# Autodesk Inventor assembly: parts assembly
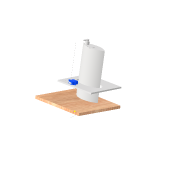
[picture p0: Inventor's stored thumbnail of the model, 180x180]
Saved by Autodesk Inventor 2021 (Build 250183000, 183)
## iProperties
Created: 2021-03-10
Part Number: parts assembly
Document SubType Name: Assembly
Designer: Dell
Author: Dell
## Documents named in this file (8)
- D:\project\parts assembly.iam
- D:\project\base.ipt
- D:\project\ir.ipt
- D:\project\Servo Motor SG90.ipt
- D:\project\arm.ipt
- D:\project\bottle support.ipt
- D:\project\container.ipt
- D:\project\rod.ipt
## Components (8 placed, 7 different names)
1. base:1 — Mate:8, Mate:9
2. ir:1 — Mate:12
3. Servo Motor SG90:1 — Mate:10, Mate:14
4. bottle support:1 — Mate:8, Mate:10
5. container:1 — Mate:9, Mate:12, Mate:13
6. arm:1 — Mate:14
7. rod:1 — Mate:13
8. rod:2
## Relationships (6: Mate 6)
- Mate:8 (50 mm): base:1 ↔ bottle support:1
- Mate:9: base:1 ↔ container:1
- Mate:10: Servo Motor SG90:1 ↔ bottle support:1
- Mate:12: ir:1 ↔ container:1
- Mate:13: container:1 ↔ rod:1
- Mate:14: Servo Motor SG90:1 ↔ arm:1
